# Autodesk Inventor assembly: POM_T5_12
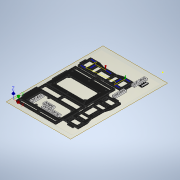
[picture p0: Inventor's stored thumbnail of the model, 180x180]
Saved by Autodesk Inventor 2020 (Build 240168000, 168)
## iProperties
Created: 2021-08-27
Part Number: POM_T5_12
Document SubType Name: Assembly
Designer: Masato
Author: Masato
## Documents named in this file (11)
- C:\Users\naoki\Documents\Inventor\CitBrains\git_clone\OpenPlatform4_1\コックピット\OpenPlatform_ver3_0\cam\POM_T5_12.iam
- C:\Users\naoki\Documents\Inventor\CitBrains\git_clone\OpenPlatform4_1\コックピット\OpenPlatform_ver3_0\cam\Disposable_Board.ipt
- C:\Users\naoki\Documents\Inventor\CitBrains\git_clone\OpenPlatform4_1\コックピット\OpenPlatform_ver3_0\UpperBody\Cockpit\Cockpit_carrier_board_frame.ipt
- C:\Users\naoki\Documents\Inventor\CitBrains\git_clone\OpenPlatform4_1\コックピット\OpenPlatform_ver3_0\UpperBody\Cockpit\Cockpit_circuit_board_frame.ipt
- C:\Users\naoki\Documents\Inventor\CitBrains\git_clone\OpenPlatform4_1\コックピット\OpenPlatform_ver3_0\JIG\Camera_side_frame_JIG.ipt
- C:\Users\naoki\Documents\Inventor\CitBrains\git_clone\OpenPlatform4_1\コックピット\OpenPlatform_ver3_0\JIG\Head_diagonal_JIG.ipt
- C:\Users\naoki\Documents\Inventor\CitBrains\git_clone\OpenPlatform4_1\コックピット\OpenPlatform_ver3_0\JIG\Head_horn_frame_JIG.ipt
- C:\Users\naoki\Documents\Inventor\CitBrains\git_clone\OpenPlatform4_1\コックピット\OpenPlatform_ver3_0\UpperBody\Trunk\Trunk_chest_frame.ipt
- C:\Users\naoki\Documents\Inventor\CitBrains\git_clone\OpenPlatform4_1\コックピット\OpenPlatform_ver3_0\JIG\Cockpit_back_frame_JIG.ipt
- C:\Users\naoki\Documents\Inventor\CitBrains\git_clone\OpenPlatform4_1\コックピット\OpenPlatform_ver3_0\JIG\Cockpit_battery_bottom_frame_JIG.ipt
- C:\Users\naoki\Documents\Inventor\CitBrains\git_clone\OpenPlatform4_1\コックピット\OpenPlatform_ver3_0\JIG\Cockpit_side_frame_JIG.ipt
## Components (11 placed, 10 different names)
1. Disposable_Board:1 — メイト:2, メイト:1, フラッシュ:1, フラッシュ:2, メイト:4, メイト:5, メイト:13, メイト:15, メイト:17, フラッシュ:4, メイト:20, メイト:22, フラッシュ:6, フラッシュ:7, フラッシュ:11, メイト:38, メイト:40, メイト:42
2. Cockpit_carrier_board_frame:1 — メイト:5, フラッシュ:4, メイト:27, メイト:28, メイト:29, 正接:1, フラッシュ:11, フラッシュ:12, メイト:35
3. Cockpit_circuit_board_frame:1 — メイト:4, フラッシュ:6, メイト:25, メイト:35, メイト:52
4. Camera_side_frame_JIG:1 — メイト:13, メイト:29, メイト:30, 正接:1
5. Head_diagonal_JIG:1 — メイト:15, メイト:30
6. Head_horn_frame_JIG:1 — メイト:17, メイト:27, メイト:28
7. Trunk_chest_frame:1 — メイト:20, メイト:25, フラッシュ:12
8. Trunk_chest_frame:2 — メイト:22, フラッシュ:7, メイト:50, メイト:51, メイト:52, メイト:53
9. Cockpit_back_frame_JIG:1 — メイト:42, メイト:53
10. Cockpit_battery_bottom_frame_JIG:1 — メイト:40, メイト:50, メイト:51, メイト:55
11. Cockpit_side_frame_JIG:1 — メイト:38, メイト:55
## Relationships (31: Mate 23, Flush 7, Tangent 1)
- メイト:2 [Mate]: Disposable_Board:1
- メイト:1 [Mate]: Disposable_Board:1
- フラッシュ:1 [Flush]: Disposable_Board:1
- フラッシュ:2 [Flush]: Disposable_Board:1
- メイト:4 [Mate]: Disposable_Board:1 ↔ Cockpit_circuit_board_frame:1
- メイト:5 [Mate]: Disposable_Board:1 ↔ Cockpit_carrier_board_frame:1
- メイト:13 [Mate]: Disposable_Board:1 ↔ Camera_side_frame_JIG:1
- メイト:15 [Mate]: Disposable_Board:1 ↔ Head_diagonal_JIG:1
- メイト:17 [Mate]: Disposable_Board:1 ↔ Head_horn_frame_JIG:1
- フラッシュ:4 [Flush] (2 mm): Disposable_Board:1 ↔ Cockpit_carrier_board_frame:1
- メイト:20 [Mate]: Disposable_Board:1 ↔ Trunk_chest_frame:1
- メイト:22 [Mate]: Disposable_Board:1 ↔ Trunk_chest_frame:2
- フラッシュ:6 [Flush] (2 mm): Disposable_Board:1 ↔ Cockpit_circuit_board_frame:1
- フラッシュ:7 [Flush] (2 mm): Disposable_Board:1 ↔ Trunk_chest_frame:2
- メイト:25 [Mate] (2.5 mm): Cockpit_circuit_board_frame:1 ↔ Trunk_chest_frame:1
- メイト:27 [Mate] (2.5 mm): Cockpit_carrier_board_frame:1 ↔ Head_horn_frame_JIG:1
- メイト:28 [Mate] (2.5 mm): Cockpit_carrier_board_frame:1 ↔ Head_horn_frame_JIG:1
- メイト:29 [Mate] (2.5 mm): Cockpit_carrier_board_frame:1 ↔ Camera_side_frame_JIG:1
- メイト:30 [Mate] (2.5 mm): Camera_side_frame_JIG:1 ↔ Head_diagonal_JIG:1
- 正接:1 [Tangent] (3 mm): Cockpit_carrier_board_frame:1 ↔ Camera_side_frame_JIG:1
- フラッシュ:11 [Flush] (2 mm): Disposable_Board:1 ↔ Cockpit_carrier_board_frame:1
- フラッシュ:12 [Flush]: Cockpit_carrier_board_frame:1 ↔ Trunk_chest_frame:1
- メイト:35 [Mate] (2.5 mm): Cockpit_carrier_board_frame:1 ↔ Cockpit_circuit_board_frame:1
- メイト:38 [Mate]: Disposable_Board:1 ↔ Cockpit_side_frame_JIG:1
- メイト:40 [Mate]: Disposable_Board:1 ↔ Cockpit_battery_bottom_frame_JIG:1
- メイト:42 [Mate]: Disposable_Board:1 ↔ Cockpit_back_frame_JIG:1
- メイト:50 [Mate] (2.5 mm): Trunk_chest_frame:2 ↔ Cockpit_battery_bottom_frame_JIG:1
- メイト:51 [Mate] (2.5 mm): Trunk_chest_frame:2 ↔ Cockpit_battery_bottom_frame_JIG:1
- メイト:52 [Mate] (2.5 mm): Cockpit_circuit_board_frame:1 ↔ Trunk_chest_frame:2
- メイト:53 [Mate] (2.5 mm): Trunk_chest_frame:2 ↔ Cockpit_back_frame_JIG:1
- メイト:55 [Mate] (2.5 mm): Cockpit_battery_bottom_frame_JIG:1 ↔ Cockpit_side_frame_JIG:1
